# Autodesk Inventor assembly: Zespół2
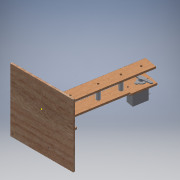
[picture p0: Inventor's stored thumbnail of the model, 180x180]
Saved by Autodesk Inventor 2017 (Build 210142000, 142)
## iProperties
Part Number: Zespół2
Material: Ogólny
Document SubType Name: Assembly
Designer: Damian
Author: Damian
## Documents named in this file (7)
- C:\Users\Damian\Documents\Inventor\Nowe\2.0\Zespół2.iam
- C:\Users\Damian\Documents\Inventor\Nowe\2.0\towerpro.ipt
- C:\Users\Damian\Documents\Inventor\Nowe\2.0\Część2.ipt
- C:\Users\Damian\Documents\Inventor\Nowe\2.0\tuleja18.ipt
- C:\Users\Damian\Documents\Inventor\Nowe\2.0\Część1.ipt
- C:\Users\Damian\Documents\Inventor\Nowe\2.0\Micro Servo 9g Arm.ipt
- C:\Users\Damian\Documents\Inventor\Nowe\2.0\podstawa.ipt
## Components (10 placed, 6 different names)
1. towerpro:1 — Sztywne:1, Wstaw:1
2. Część2:1 — Sztywne:1, Sztywne:2, Sztywne:3, Sztywne:4, Obrotowe:1
3. Część1:1 — Obrotowe:1, Wstaw:3, Obrotowe:3
4. tuleja18:1 — Sztywne:2, Obrotowe:3
5. tuleja18:2 — Sztywne:3
6. tuleja18:3 — Sztywne:4
7. Micro Servo 9g Arm:1 — Wstaw:1
8. podstawa:1 — Obrotowe:2, Wstaw:3
9. towerpro:2 — Obrotowe:2, Wstaw:2
10. Micro Servo 9g Arm:2 — Wstaw:2
## Relationships (10: WeldJoint 4, Insert 3, RevoluteJoint 3)
- Sztywne:1 [WeldJoint] (-4 mm): towerpro:1 ↔ Część2:1
- Sztywne:2 [WeldJoint]: Część2:1 ↔ tuleja18:1
- Sztywne:3 [WeldJoint]: Część2:1 ↔ tuleja18:2
- Sztywne:4 [WeldJoint]: Część2:1 ↔ tuleja18:3
- Wstaw:1 [Insert]: towerpro:1 ↔ Micro Servo 9g Arm:1
- Obrotowe:1 [RevoluteJoint] (18 mm): Część2:1 ↔ Część1:1
- Obrotowe:2 [RevoluteJoint] (4 mm): podstawa:1 ↔ towerpro:2
- Wstaw:2 [Insert]: towerpro:2 ↔ Micro Servo 9g Arm:2
- Wstaw:3 [Insert]: Część1:1 ↔ podstawa:1
- Obrotowe:3 [RevoluteJoint]: Część1:1 ↔ tuleja18:1
